# Autodesk Inventor assembly: sideassembly(sa)
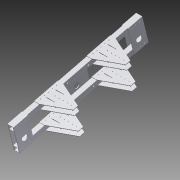
[picture p0: Inventor's stored thumbnail of the model, 180x180]
Saved by Autodesk Inventor 2015 (Build 190159000, 159)
## iProperties
Created: 2015-10-03
Part Number: sideassembly(sa)
Document SubType Name: Assembly
Designer: elilitwack
Mass: 2214.44 g
Surface Area: 7372.09 cm^2
Volume: 820.163 cm^3
Density: 2.7 g/cm^3
Author: elilitwack
## Documents named in this file (5)
- C:\Users\elilitwack\Documents\2015 Offseason Chassis\West Coast Chassis Fall 2015 - iLogic\sideassembly(sa).iam
- C:\Users\elilitwack\Documents\2015 Offseason Chassis\West Coast Chassis Fall 2015 - iLogic\sidetube(st.ipt
- C:\Users\elilitwack\Documents\2015 Offseason Chassis\West Coast Chassis Fall 2015 - iLogic\bearingplate(bp).ipt
- C:\Users\elilitwack\Documents\2015 Offseason Chassis\West Coast Chassis Fall 2015 - iLogic\gearboxbearingplate(gbpb).ipt
- C:\Users\elilitwack\Documents\2015 Offseason Chassis\West Coast Chassis Fall 2015 - iLogic\traingle_bracket(tb).ipt
## Components (15 placed, 4 different names)
1. sidetube(st:1 — Mate:9, Mate:10, Mate:11, Mate:12, Mate:13, Mate:14, Mate:27, Mate:28, Mate:29, Mate:33, Mate:34, Mate:35, Mate:36, Mate:37, Mate:38, Mate:45, Mate:46, Mate:47, Mate:48, Mate:49, Mate:50, Mate:57, Mate:58, Mate:59, Mate:60, Mate:61, Mate:62
2. sidetube(st:2 — Mate:15, Mate:16, Mate:17, Mate:18, Mate:19, Mate:20, Mate:51, Mate:52, Mate:53, Mate:54, Mate:55, Mate:56, Mate:63, Mate:64, Mate:65, Mate:66, Mate:67, Mate:68
3. bearingplate(bp):1 — Mate:11, Mate:12, Mate:14, Mate:17, Mate:18, Mate:19
4. bearingplate(bp):2 — Mate:9, Mate:10, Mate:13, Mate:15, Mate:16, Mate:20
5. gearboxbearingplate(gbpb):1 — Mate:27, Mate:28, Mate:29
6. bearingplate(bp):3 — Mate:36, Mate:37, Mate:38
7. bearingplate(bp):4 — Mate:33, Mate:34, Mate:35
8. traingle_bracket(tb):1 — Mate:45, Mate:46, Mate:47
9. traingle_bracket(tb):2 — Mate:57, Mate:58, Mate:59
10. traingle_bracket(tb):3 — Mate:60, Mate:61, Mate:62
11. traingle_bracket(tb):4 — Mate:48, Mate:49, Mate:50
12. traingle_bracket(tb):5 — Mate:51, Mate:52, Mate:53
13. traingle_bracket(tb):6 — Mate:54, Mate:55, Mate:56
14. traingle_bracket(tb):7 — Mate:63, Mate:64, Mate:65
15. traingle_bracket(tb):8 — Mate:66, Mate:67, Mate:68
## Relationships (45: Mate 45)
- Mate:9: sidetube(st:1 ↔ bearingplate(bp):2
- Mate:10: sidetube(st:1 ↔ bearingplate(bp):2
- Mate:11: sidetube(st:1 ↔ bearingplate(bp):1
- Mate:12: sidetube(st:1 ↔ bearingplate(bp):1
- Mate:13: sidetube(st:1 ↔ bearingplate(bp):2
- Mate:14: sidetube(st:1 ↔ bearingplate(bp):1
- Mate:15: sidetube(st:2 ↔ bearingplate(bp):2
- Mate:16: sidetube(st:2 ↔ bearingplate(bp):2
- Mate:17: sidetube(st:2 ↔ bearingplate(bp):1
- Mate:18: sidetube(st:2 ↔ bearingplate(bp):1
- Mate:19: sidetube(st:2 ↔ bearingplate(bp):1
- Mate:20: sidetube(st:2 ↔ bearingplate(bp):2
- Mate:27: sidetube(st:1 ↔ gearboxbearingplate(gbpb):1
- Mate:28: sidetube(st:1 ↔ gearboxbearingplate(gbpb):1
- Mate:29: sidetube(st:1 ↔ gearboxbearingplate(gbpb):1
- Mate:33: sidetube(st:1 ↔ bearingplate(bp):4
- Mate:34: sidetube(st:1 ↔ bearingplate(bp):4
- Mate:35: sidetube(st:1 ↔ bearingplate(bp):4
- Mate:36: sidetube(st:1 ↔ bearingplate(bp):3
- Mate:37: sidetube(st:1 ↔ bearingplate(bp):3
- Mate:38: sidetube(st:1 ↔ bearingplate(bp):3
- Mate:45: sidetube(st:1 ↔ traingle_bracket(tb):1
- Mate:46: sidetube(st:1 ↔ traingle_bracket(tb):1
- Mate:47: sidetube(st:1 ↔ traingle_bracket(tb):1
- Mate:48: sidetube(st:1 ↔ traingle_bracket(tb):4
- Mate:49: sidetube(st:1 ↔ traingle_bracket(tb):4
- Mate:50: sidetube(st:1 ↔ traingle_bracket(tb):4
- Mate:51: sidetube(st:2 ↔ traingle_bracket(tb):5
- Mate:52: sidetube(st:2 ↔ traingle_bracket(tb):5
- Mate:53: sidetube(st:2 ↔ traingle_bracket(tb):5
- Mate:54: sidetube(st:2 ↔ traingle_bracket(tb):6
- Mate:55: sidetube(st:2 ↔ traingle_bracket(tb):6
- Mate:56: sidetube(st:2 ↔ traingle_bracket(tb):6
- Mate:57: sidetube(st:1 ↔ traingle_bracket(tb):2
- Mate:58: sidetube(st:1 ↔ traingle_bracket(tb):2
- Mate:59: sidetube(st:1 ↔ traingle_bracket(tb):2
- Mate:60: sidetube(st:1 ↔ traingle_bracket(tb):3
- Mate:61: sidetube(st:1 ↔ traingle_bracket(tb):3
- Mate:62: sidetube(st:1 ↔ traingle_bracket(tb):3
- Mate:63: sidetube(st:2 ↔ traingle_bracket(tb):7
- Mate:64: sidetube(st:2 ↔ traingle_bracket(tb):7
- Mate:65: sidetube(st:2 ↔ traingle_bracket(tb):7
- Mate:66: sidetube(st:2 ↔ traingle_bracket(tb):8
- Mate:67: sidetube(st:2 ↔ traingle_bracket(tb):8
- Mate:68: sidetube(st:2 ↔ traingle_bracket(tb):8
